# Autodesk Inventor assembly: 20
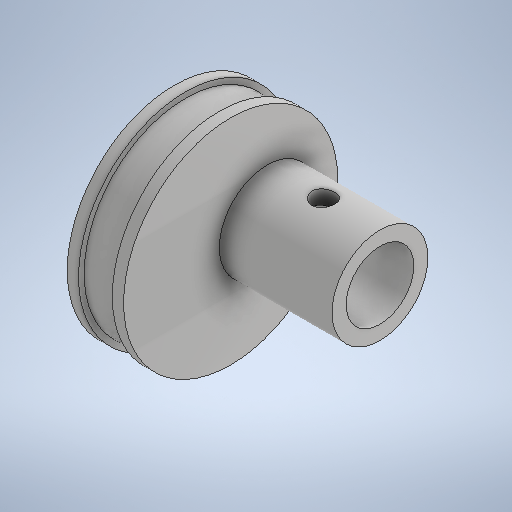
[picture p0: Inventor's stored thumbnail of the model, 512x512]
Saved by Autodesk Inventor 2025.1 (Build 291241000, 241)
## iProperties
Created: 2024-09-13
Part Number: 20
Document SubType Name: Assembly
Designer: ffogue
Author: ffogue
## Documents named in this file (4)
- C:\Users\ffogue\Documents\Inventor\Single cylinder Steam Engine\20.iam
- C:\Users\ffogue\Documents\Inventor\Single cylinder Steam Engine\20.1.ipt
- C:\Users\ffogue\Documents\Inventor\Single cylinder Steam Engine\20.2.ipt
- C:\Users\ffogue\Documents\Inventor\Single cylinder Steam Engine\20.3.ipt
## Components (4 placed, 3 different names)
1. 20.2:1 — Mate:1, Insert:1
2. 20.1:2 — Mate:1, Insert:1, Mate:2, Insert:2
3. 20.2:2 — Mate:2, Insert:2, Mate:3, Flush:1
4. 20.3:1 — Mate:3, Flush:1
## Relationships (6: Mate 3, Insert 2, Flush 1)
- Mate:1: 20.2:1 ↔ 20.1:2
- Insert:1: 20.2:1 ↔ 20.1:2
- Mate:2: 20.1:2 ↔ 20.2:2
- Insert:2: 20.1:2 ↔ 20.2:2
- Mate:3: 20.2:2 ↔ 20.3:1
- Flush:1 (-0.5 mm): 20.2:2 ↔ 20.3:1
